# Autodesk Inventor assembly: 装配-载板上盖
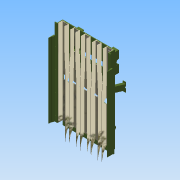
[picture p0: Inventor's stored thumbnail of the model, 180x180]
Saved by Autodesk Inventor 2015 (Build 190159000, 159)
## iProperties
Created: 2017-05-23
Part Number: 装配-载板上盖
Document SubType Name: Assembly
Designer: Administrator
Author: Administrator
## Documents named in this file (6)
- C:\Users\Administrator\Desktop\毕设改\装配-载板上盖.iam
- C:\Users\Administrator\Desktop\毕设改\载板上盖.ipt
- C:\Users\Administrator\Desktop\毕设改\载板下弹片固定螺丝.ipt
- C:\Users\Administrator\Desktop\毕设改\载板下弹片内3.ipt
- C:\Users\Administrator\Desktop\毕设改\载板下弹片右.ipt
- C:\Users\Administrator\Desktop\毕设改\载板下弹片左.ipt
## Components (16 placed, 5 different names)
1. 载板上盖:1 — 插入:1, 插入:2, 插入:4, 插入:5, 插入:6, 插入:7, 插入:8, 插入:9, 插入:10, 插入:11
2. 载板下弹片固定螺丝:1 — 插入:3
3. 载板下弹片内3:1 — 插入:4, 插入:8, 插入:12, 插入:17
4. 载板下弹片右:1 — 插入:1, 插入:2, 插入:3, 插入:16
5. 载板下弹片左:1 — 插入:7, 插入:11, 插入:15, 插入:20
6. 载板下弹片内3:2 — 插入:5, 插入:9, 插入:13, 插入:18
7. 载板下弹片内3:3 — 插入:6, 插入:10, 插入:14, 插入:19
8. 载板下弹片固定螺丝:2 — 插入:12
9. 载板下弹片固定螺丝:3 — 插入:13
10. 载板下弹片固定螺丝:4 — 插入:14
11. 载板下弹片固定螺丝:5 — 插入:15
12. 载板下弹片固定螺丝:6 — 插入:16
13. 载板下弹片固定螺丝:7 — 插入:17
14. 载板下弹片固定螺丝:8 — 插入:18
15. 载板下弹片固定螺丝:9 — 插入:19
16. 载板下弹片固定螺丝:10 — 插入:20
## Relationships (20: Insert 20)
- 插入:1 [Insert]: 载板上盖:1 ↔ 载板下弹片右:1
- 插入:2 [Insert]: 载板上盖:1 ↔ 载板下弹片右:1
- 插入:3 [Insert]: 载板下弹片固定螺丝:1 ↔ 载板下弹片右:1
- 插入:4 [Insert]: 载板上盖:1 ↔ 载板下弹片内3:1
- 插入:5 [Insert]: 载板上盖:1 ↔ 载板下弹片内3:2
- 插入:6 [Insert]: 载板上盖:1 ↔ 载板下弹片内3:3
- 插入:7 [Insert]: 载板上盖:1 ↔ 载板下弹片左:1
- 插入:8 [Insert]: 载板上盖:1 ↔ 载板下弹片内3:1
- 插入:9 [Insert]: 载板上盖:1 ↔ 载板下弹片内3:2
- 插入:10 [Insert]: 载板上盖:1 ↔ 载板下弹片内3:3
- 插入:11 [Insert]: 载板上盖:1 ↔ 载板下弹片左:1
- 插入:12 [Insert]: 载板下弹片内3:1 ↔ 载板下弹片固定螺丝:2
- 插入:13 [Insert]: 载板下弹片内3:2 ↔ 载板下弹片固定螺丝:3
- 插入:14 [Insert]: 载板下弹片内3:3 ↔ 载板下弹片固定螺丝:4
- 插入:15 [Insert]: 载板下弹片左:1 ↔ 载板下弹片固定螺丝:5
- 插入:16 [Insert]: 载板下弹片右:1 ↔ 载板下弹片固定螺丝:6
- 插入:17 [Insert]: 载板下弹片内3:1 ↔ 载板下弹片固定螺丝:7
- 插入:18 [Insert]: 载板下弹片内3:2 ↔ 载板下弹片固定螺丝:8
- 插入:19 [Insert]: 载板下弹片内3:3 ↔ 载板下弹片固定螺丝:9
- 插入:20 [Insert]: 载板下弹片左:1 ↔ 载板下弹片固定螺丝:10
